# Autodesk Inventor assembly: V-Slot Gantry Kit - 20mm
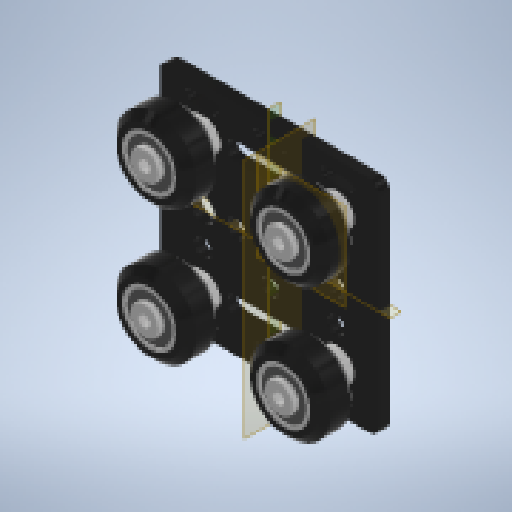
[picture p0: Inventor's stored thumbnail of the model, 512x512]
Saved by Autodesk Inventor 2023 (Build 270158000, 158)
## iProperties
Created: 2019-10-15
Part Number: V-Slot Gantry Kit - 20mm
Document SubType Name: Assembly
Designer: Felix
Sending System: Autodesk Translation Framework v8.6.0.1094
Preprocessor: ST-DEVELOPER v18
Title: /Users/ayahni/Desktop/V-Slot Gantry Kit - 20mm.step
## Documents named in this file (10)
- D:\Programmieren\PineapplePenPlotter\Inventor\StoreBought\4022_20220624140806_V-Slot Gantry Kit - 20mm.iam
- D:\Programmieren\PineapplePenPlotter\Inventor\StoreBought\V-Slot Gantry Plate 20mm v1.ipt
- D:\Programmieren\PineapplePenPlotter\Inventor\StoreBought\Low Profile Screw M5 v1.ipt
- D:\Programmieren\PineapplePenPlotter\Inventor\StoreBought\Nylon Insert Lock Nut M5 v1.ipt
- D:\Programmieren\PineapplePenPlotter\Inventor\StoreBought\Aluminum Spacer 6mm v1.ipt
- D:\Programmieren\PineapplePenPlotter\Inventor\StoreBought\Eccentric Spacer 6mm v1.ipt
- D:\Programmieren\PineapplePenPlotter\Inventor\StoreBought\Ball Bearing 5 x 16 x 5 v1.ipt
- D:\Programmieren\PineapplePenPlotter\Inventor\StoreBought\Precision Shim 8 x 5 x 1 v1.ipt
- D:\Programmieren\PineapplePenPlotter\Inventor\StoreBought\Xtreme Solid V Wheel v1.ipt
- D:\Programmieren\PineapplePenPlotter\Inventor\plotter_try_2\PlaneHelpPart.ipt
## Components (30 placed, 9 different names)
1. V-Slot Gantry Plate 20mm v1:1 — Flush:1, Flush:2, Angle:2, Mate:2, Mate:3, Angle:3, Angle:4
2. Low Profile Screw M5 v1:1
3. Nylon Insert Lock Nut M5 v1:1 — Angle:1
4. Aluminum Spacer 6mm v1:1
5. Eccentric Spacer 6mm v1:1
6. Ball Bearing 5 x 16 x 5 v1:1
7. Precision Shim 8 x 5 x 1 v1:1
8. Ball Bearing 5 x 16 x 5 v1:2
9. Ball Bearing 5 x 16 x 5 v1:3
10. Precision Shim 8 x 5 x 1 v1:2
11. Ball Bearing 5 x 16 x 5 v1:4
12. Nylon Insert Lock Nut M5 v1:2
13. Low Profile Screw M5 v1:2
14. Low Profile Screw M5 v1:3
15. Nylon Insert Lock Nut M5 v1:3
16. Ball Bearing 5 x 16 x 5 v1:5
17. Precision Shim 8 x 5 x 1 v1:3
18. Ball Bearing 5 x 16 x 5 v1:6
19. Eccentric Spacer 6mm v1:2
20. Low Profile Screw M5 v1:4
21. Nylon Insert Lock Nut M5 v1:4
22. Aluminum Spacer 6mm v1:2
23. Ball Bearing 5 x 16 x 5 v1:7
24. Precision Shim 8 x 5 x 1 v1:4
25. Ball Bearing 5 x 16 x 5 v1:8 — Symmetry:1
26. Xtreme Solid V Wheel v1:1 — Tangent:1, Symmetry:1
27. Xtreme Solid V Wheel v1:2
28. Xtreme Solid V Wheel v1:3
29. Xtreme Solid V Wheel v1:4
30. PlaneHelpPart:1 — Flush:1, Flush:2, Mate:1
## Relationships (14: Mate 6, Angle 4, Flush 2, Tangent 1, Symmetry 1)
- Angle:1 (0 deg): Nylon Insert Lock Nut M5 v1:1
- Tangent:1: Xtreme Solid V Wheel v1:1
- Symmetry:1: Ball Bearing 5 x 16 x 5 v1:8 ↔ Xtreme Solid V Wheel v1:1
- Flush:1: V-Slot Gantry Plate 20mm v1:1 ↔ PlaneHelpPart:1
- Flush:2: V-Slot Gantry Plate 20mm v1:1 ↔ PlaneHelpPart:1
- Mate:1: PlaneHelpPart:1
- Angle:2 (0 deg): V-Slot Gantry Plate 20mm v1:1
- Mate:2: V-Slot Gantry Plate 20mm v1:1
- Mate:3: V-Slot Gantry Plate 20mm v1:1
- Mate:4
- Mate:5
- Angle:3 (0 deg): V-Slot Gantry Plate 20mm v1:1
- Mate:6
- Angle:4 (0 deg): V-Slot Gantry Plate 20mm v1:1
